# Autodesk Inventor assembly: Durometer_Assembly
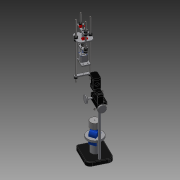
[picture p0: Inventor's stored thumbnail of the model, 180x180]
Saved by Autodesk Inventor 2015 (Build 190159000, 159)
## iProperties
Created: 2014-12-16
Part Number: Durometer_Assembly
Document SubType Name: Assembly
Designer: amarschn
Author: amarschn
## Documents named in this file (7)
- C:\Users\Drew\Dropbox\Durometer\Durometer_Assembly\Durometer_Assembly.iam
- C:\Users\Drew\Dropbox\Durometer\Durometer_Assembly\Durometer_Base.ipt
- C:\Users\Drew\Dropbox\Durometer\Durometer_Assembly\Durometer_Slide_Shaft.ipt
- C:\Users\Drew\Dropbox\Durometer\Durometer_Assembly\Durometer_Platform.ipt
- C:\Users\Drew\Dropbox\Durometer\Durometer_Assembly\Durometer_Slide_Fixture.iam
- C:\Users\Drew\Dropbox\Durometer\Durometer_Assembly\Durometer_Lead_Screw_Fixture.iam
- C:\Users\Drew\Dropbox\Durometer\Durometer_Assembly\Durometer_Vertical_Lead_Screw_Assembly.iam
## Components (6 placed, 6 different names)
1. Durometer_Base:1 — Insert:1, Flush:1, Mate:1
2. Durometer_Slide_Shaft:1 — Insert:1, Mate:2, Flush:2
3. Durometer_Platform:1 — Flush:1, Mate:1
4. Durometer_Slide_Fixture:1 [sub-assembly] — Mate:2, Flush:2, Mate:3, Flush:3, Mate:4, Flush:4
5. Durometer_Lead_Screw_Fixture:1 [sub-assembly] — Mate:3, Flush:3, Mate:4
6. Durometer_Vertical_Lead_Screw_Assembly:1 [sub-assembly] — Flush:4
## Relationships (9: Flush 4, Mate 4, Insert 1)
- Insert:1: Durometer_Base:1 ↔ Durometer_Slide_Shaft:1
- Flush:1: Durometer_Base:1 ↔ Durometer_Platform:1
- Mate:1: Durometer_Base:1 ↔ Durometer_Platform:1
- Mate:2: Durometer_Slide_Shaft:1 ↔ Durometer_Slide_Fixture:1
- Flush:2 (-20 mm): Durometer_Slide_Shaft:1 ↔ Durometer_Slide_Fixture:1
- Mate:3: Durometer_Slide_Fixture:1 ↔ Durometer_Lead_Screw_Fixture:1
- Flush:3: Durometer_Slide_Fixture:1 ↔ Durometer_Lead_Screw_Fixture:1
- Mate:4: Durometer_Slide_Fixture:1 ↔ Durometer_Lead_Screw_Fixture:1
- Flush:4: Durometer_Slide_Fixture:1 ↔ Durometer_Vertical_Lead_Screw_Assembly:1
